# Autodesk Inventor assembly: Столб_переда_корпуса_2.0_MIR
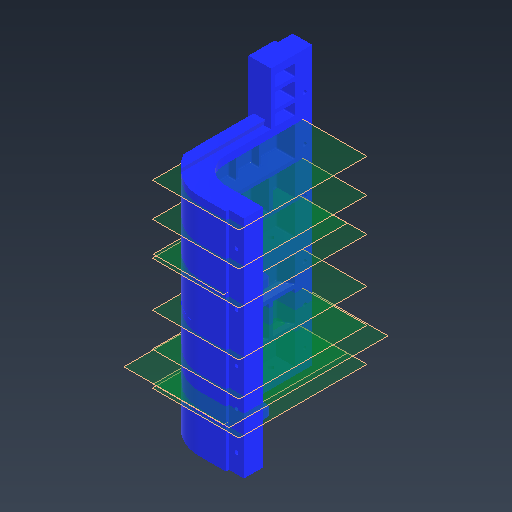
[picture p0: Inventor's stored thumbnail of the model, 512x512]
Saved by Autodesk Inventor 2023.2 (Build 272271030, 271C)
## iProperties
Created: 2025-10-02
Part Number: Столб_переда_корпуса_2.0_MIR
Document SubType Name: Assembly
Designer: Олег Коноваленко
Author: Олег Коноваленко
## Documents named in this file (3)
- D:\!Rover\Rover\Rover_construction\Столб_переда_корпуса_2.0_MIR.iam
- D:\!Rover\Rover\Rover_construction\Столб_версия_2.0_MIR.ipt
- D:\!Rover\Rover\Rover_construction\Верхняя_ часть_переднего_столба_2.0_MIR.ipt
## Components (2 placed, 2 different names)
1. Столб_версия_2.0_MIR:1 — Заподлицо:2, Заподлицо:1, Совмещение:1
2. Верхняя_ часть_переднего_столба_2.0_MIR:1 — Заподлицо:2, Заподлицо:1, Совмещение:1
## Relationships (3: Flush 2, Mate 1)
- Заподлицо:2 [Flush]: Столб_версия_2.0_MIR:1 ↔ Верхняя_ часть_переднего_столба_2.0_MIR:1
- Заподлицо:1 [Flush]: Столб_версия_2.0_MIR:1 ↔ Верхняя_ часть_переднего_столба_2.0_MIR:1
- Совмещение:1 [Mate]: Столб_версия_2.0_MIR:1 ↔ Верхняя_ часть_переднего_столба_2.0_MIR:1
